# Autodesk Inventor assembly: linear slide
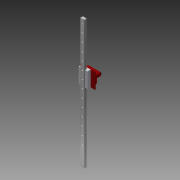
[picture p0: Inventor's stored thumbnail of the model, 180x180]
Saved by Autodesk Inventor 2015 SP1 (Build 190203100, 203)
## iProperties
Created: 2015-02-03
Part Number: linear slide
Document SubType Name: Assembly
Designer: Joseph
Author: Joseph
## Documents named in this file (4)
- C:\Users\Joseph\Documents\GitHub\mchp_kossel\Printer\linear slide.iam
- C:\Users\Joseph\Documents\GitHub\mchp_kossel\Printer\slide.ipt
- C:\Users\Joseph\Documents\GitHub\mchp_kossel\Printer\Carraige.ipt
- C:\Users\Joseph\Documents\GitHub\mchp_kossel\Printer\slide rail.ipt
## Components (3 placed, 3 different names)
1. slide:1 — Flush:1, Planar:1, Mate:2
2. Carraige:1 — Flush:1
3. slide rail:1 — Planar:1, Mate:2
## Relationships (3: Flush 1, PlanarJoint 1, Mate 1)
- Flush:1: slide:1 ↔ Carraige:1
- Planar:1: slide:1 ↔ slide rail:1
- Mate:2: slide:1 ↔ slide rail:1
